# Autodesk Inventor assembly: 000-base_wheel-v2
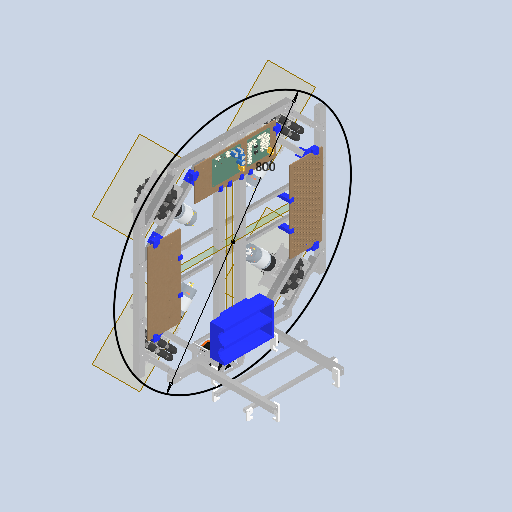
[picture p0: Inventor's stored thumbnail of the model, 512x512]
Saved by Autodesk Inventor 2025.2 (Build 292293000, 293)
## iProperties
Created: 2025-01-06
Part Number: 000-base_wheel-v2
Document SubType Name: Assembly
Designer: haruy
Mass: 4431.15 g
Surface Area: 15153.5 cm^2
Volume: 1600.59 cm^3
Density: 2.76846 g/cm^3
Author: haruy
## Documents named in this file (61)
- C:\Users\haruy\Documents\ロボコン\NHK2025\cad\nagahisa\base_weel\000-base_wheel-v2.iam
- C:\Users\haruy\Documents\ロボコン\NHK2025\cad\nagahisa\base_weel\base_weel-v2-ASP-Base.ipt
- C:\Users\haruy\Documents\ロボコン\NHK2025\cad\nagahisa\base_weel\takagi_weel\Workspaces\作業スペース\takagi\omuni_wheel_ver3.0\parts\omu_al_jo_1.ipt
- C:\Users\haruy\Documents\ロボコン\NHK2025\cad\nagahisa\base_weel\takagi_weel\Workspaces\作業スペース\takagi\omuni_wheel_ver3.0\parts\omu_al_jo_3.ipt
- C:\Users\haruy\Documents\ロボコン\NHK2025\cad\nagahisa\base_weel\takagi_weel\Workspaces\作業スペース\takagi\omuni_wheel_ver3.0\parts\frequently used parts\モーター\RS775\rs775_4.iam
- C:\Users\haruy\Documents\ロボコン\NHK2025\cad\nagahisa\base_weel\takagi_weel\Workspaces\作業スペース\takagi\omuni_wheel_ver3.0\parts\frequently used parts\セットカラー\SSCSP12-10\SSCSP12-10.iam
- C:\Users\haruy\Documents\ロボコン\NHK2025\cad\nagahisa\base_weel\takagi_weel\Workspaces\作業スペース\takagi\omuni_wheel_ver3.0\parts\omu_al_jo_2.ipt
- C:\Users\haruy\Documents\ロボコン\NHK2025\cad\nagahisa\base_weel\takagi_weel\Workspaces\作業スペース\takagi\omuni_wheel_ver3.0\parts\omu_sh_jo_2.ipt
- C:\Users\haruy\Documents\ロボコン\NHK2025\cad\nagahisa\base_weel\takagi_weel\Workspaces\作業スペース\takagi\omuni_wheel_ver3.0\parts\omu_sh_jo_3.ipt
- C:\Users\haruy\Documents\ロボコン\NHK2025\cad\nagahisa\base_weel\takagi_weel\Workspaces\作業スペース\takagi\omuni_wheel_ver3.0\parts\frequently used parts\ベアリング\B6201ZZNR\bearingB6201ZZNR.ipt
- C:\Users\haruy\Documents\ロボコン\NHK2025\cad\nagahisa\base_weel\takagi_weel\Workspaces\作業スペース\takagi\omuni_wheel_ver3.0\parts\frequently used parts\タイヤ\omni wheel\100mm wheel\100mm omuniwheel_MIR1.iam
- C:\Users\haruy\Documents\ロボコン\NHK2025\cad\nagahisa\base_weel\takagi_weel\Workspaces\作業スペース\takagi\omuni_wheel_ver3.0\parts\omu_al_jo_1_MIR2.ipt
- C:\Users\haruy\Documents\ロボコン\NHK2025\cad\nagahisa\base_weel\takagi_weel\Workspaces\作業スペース\takagi\omuni_wheel_ver3.0\parts\omu_al_jo_3_MIR2.ipt
- C:\Users\haruy\Documents\ロボコン\NHK2025\cad\nagahisa\base_weel\takagi_weel\Workspaces\作業スペース\takagi\omuni_wheel_ver3.0\parts\frequently used parts\モーター\RS775\rs775_4_MIR2.iam
- C:\Users\haruy\Documents\ロボコン\NHK2025\cad\nagahisa\base_weel\takagi_weel\Workspaces\作業スペース\takagi\omuni_wheel_ver3.0\parts\frequently used parts\セットカラー\SSCSP12-10\SSCSP12-10_MIR2.iam
- C:\Users\haruy\Documents\ロボコン\NHK2025\cad\nagahisa\base_weel\takagi_weel\Workspaces\作業スペース\takagi\omuni_wheel_ver3.0\parts\omu_al_jo_2_MIR2.ipt
- C:\Users\haruy\Documents\ロボコン\NHK2025\cad\nagahisa\base_weel\takagi_weel\Workspaces\作業スペース\takagi\omuni_wheel_ver3.0\parts\omu_sh_jo_2_MIR2.ipt
- C:\Users\haruy\Documents\ロボコン\NHK2025\cad\nagahisa\base_weel\takagi_weel\Workspaces\作業スペース\takagi\omuni_wheel_ver3.0\parts\omu_sh_jo_3_MIR2.ipt
- C:\Users\haruy\Documents\ロボコン\NHK2025\cad\nagahisa\base_weel\takagi_weel\Workspaces\作業スペース\takagi\omuni_wheel_ver3.0\parts\frequently used parts\ベアリング\B6201ZZNR\bearingB6201ZZNR_MIR2.ipt
- C:\Users\haruy\Documents\ロボコン\NHK2025\cad\nagahisa\base_weel\takagi_weel\Workspaces\作業スペース\takagi\omuni_wheel_ver3.0\parts\frequently used parts\タイヤ\omni wheel\100mm wheel\100mm omuniwheel_MIR1_MIR.iam
- C:\Users\haruy\Documents\ロボコン\NHK2025\cad\nagahisa\base_weel\takagi_weel\Workspaces\作業スペース\takagi\omuni_wheel_ver3.0\parts\omu_al_jo_1_MIR3.ipt
- C:\Users\haruy\Documents\ロボコン\NHK2025\cad\nagahisa\base_weel\takagi_weel\Workspaces\作業スペース\takagi\omuni_wheel_ver3.0\parts\omu_al_jo_3_MIR3.ipt
- C:\Users\haruy\Documents\ロボコン\NHK2025\cad\nagahisa\base_weel\takagi_weel\Workspaces\作業スペース\takagi\omuni_wheel_ver3.0\parts\frequently used parts\モーター\RS775\rs775_4_MIR3.iam
- C:\Users\haruy\Documents\ロボコン\NHK2025\cad\nagahisa\base_weel\takagi_weel\Workspaces\作業スペース\takagi\omuni_wheel_ver3.0\parts\frequently used parts\セットカラー\SSCSP12-10\SSCSP12-10_MIR3.iam
- C:\Users\haruy\Documents\ロボコン\NHK2025\cad\nagahisa\base_weel\takagi_weel\Workspaces\作業スペース\takagi\omuni_wheel_ver3.0\parts\omu_al_jo_2_MIR3.ipt
- C:\Users\haruy\Documents\ロボコン\NHK2025\cad\nagahisa\base_weel\takagi_weel\Workspaces\作業スペース\takagi\omuni_wheel_ver3.0\parts\omu_sh_jo_2_MIR3.ipt
- C:\Users\haruy\Documents\ロボコン\NHK2025\cad\nagahisa\base_weel\takagi_weel\Workspaces\作業スペース\takagi\omuni_wheel_ver3.0\parts\omu_sh_jo_3_MIR3.ipt
- C:\Users\haruy\Documents\ロボコン\NHK2025\cad\nagahisa\base_weel\takagi_weel\Workspaces\作業スペース\takagi\omuni_wheel_ver3.0\parts\frequently used parts\ベアリング\B6201ZZNR\bearingB6201ZZNR_MIR3.ipt
- C:\Users\haruy\Documents\ロボコン\NHK2025\cad\nagahisa\base_weel\takagi_weel\Workspaces\作業スペース\takagi\omuni_wheel_ver3.0\parts\frequently used parts\タイヤ\omni wheel\100mm wheel\100mm omuniwheel_MIR1_MIR1.iam
- C:\Users\haruy\Documents\ロボコン\NHK2025\cad\nagahisa\base_weel\takagi_weel\Workspaces\作業スペース\takagi\omuni_wheel_ver3.0\parts\omu_al_jo_1_MIR2_MIR.ipt
- C:\Users\haruy\Documents\ロボコン\NHK2025\cad\nagahisa\base_weel\takagi_weel\Workspaces\作業スペース\takagi\omuni_wheel_ver3.0\parts\omu_al_jo_3_MIR2_MIR.ipt
- C:\Users\haruy\Documents\ロボコン\NHK2025\cad\nagahisa\base_weel\takagi_weel\Workspaces\作業スペース\takagi\omuni_wheel_ver3.0\parts\frequently used parts\モーター\RS775\rs775_4_MIR2_MIR.iam
- C:\Users\haruy\Documents\ロボコン\NHK2025\cad\nagahisa\base_weel\takagi_weel\Workspaces\作業スペース\takagi\omuni_wheel_ver3.0\parts\frequently used parts\セットカラー\SSCSP12-10\SSCSP12-10_MIR2_MIR.iam
- C:\Users\haruy\Documents\ロボコン\NHK2025\cad\nagahisa\base_weel\takagi_weel\Workspaces\作業スペース\takagi\omuni_wheel_ver3.0\parts\omu_al_jo_2_MIR2_MIR.ipt
- C:\Users\haruy\Documents\ロボコン\NHK2025\cad\nagahisa\base_weel\takagi_weel\Workspaces\作業スペース\takagi\omuni_wheel_ver3.0\parts\omu_sh_jo_2_MIR2_MIR.ipt
- C:\Users\haruy\Documents\ロボコン\NHK2025\cad\nagahisa\base_weel\takagi_weel\Workspaces\作業スペース\takagi\omuni_wheel_ver3.0\parts\omu_sh_jo_3_MIR2_MIR.ipt
- C:\Users\haruy\Documents\ロボコン\NHK2025\cad\nagahisa\base_weel\takagi_weel\Workspaces\作業スペース\takagi\omuni_wheel_ver3.0\parts\frequently used parts\ベアリング\B6201ZZNR\bearingB6201ZZNR_MIR2_MIR.ipt
- C:\Users\haruy\Documents\ロボコン\NHK2025\cad\nagahisa\base_weel\takagi_weel\Workspaces\作業スペース\takagi\omuni_wheel_ver3.0\parts\frequently used parts\タイヤ\omni wheel\100mm wheel\100mm omuniwheel_MIR1_MIR_MIR.iam
- C:\Users\haruy\Documents\ロボコン\NHK2025\cad\nagahisa\base_weel\base_weel-v2-Plate-3.ipt
- C:\Users\haruy\Documents\ロボコン\NHK2025\cad\nagahisa\base_weel\base_weel-v2-Plate-3_MIR.ipt
- C:\Users\haruy\Documents\ロボコン\NHK2025\cad\nagahisa\base_weel\base_weel-v2-Plate-3_MIR1.ipt
- C:\Users\haruy\Documents\ロボコン\NHK2025\cad\nagahisa\base_weel\base_weel-v2-Plate-3_MIR_MIR.ipt
- C:\Users\haruy\Documents\ロボコン\NHK2025\cad\nagahisa\base_weel\base_weel-v2-Plate-4.ipt
- C:\Users\haruy\Documents\ロボコン\NHK2025\cad\nagahisa\base_weel\base_weel-v2-Plate-5.ipt
- C:\Users\haruy\Documents\ロボコン\NHK2025\cad\000_parts\センサー\LiDAR_true.iam
- C:\Users\haruy\Documents\ロボコン\NHK2025\cad\nagahisa\base_weel\base_weel-v1-Shaft-lider-spesa.ipt
- C:\Users\haruy\Documents\ロボコン\NHK2025\cad\nagahisa\base_weel\base_weel-v2-Plate-6.ipt
- C:\Users\haruy\Documents\ロボコン\NHK2025\cad\nagahisa\base_weel\base_weel-v2-Plate-7.ipt
- C:\Users\haruy\Documents\ロボコン\NHK2025\cad\nagahisa\base_weel\base_weel-v2-3DP-C-F-1.ipt
- C:\Users\haruy\Documents\ロボコン\NHK2025\cad\nagahisa\base_weel\base_weel-v2-3DP-C-F-1_MIR.ipt
- C:\Users\haruy\Documents\ロボコン\NHK2025\cad\nagahisa\base_weel\base_weel-v2-MDF-1.ipt
- C:\Users\haruy\Documents\ロボコン\NHK2025\cad\000_parts\回路関連\DCMD_Controller.ipt
- C:\Users\haruy\Documents\ロボコン\NHK2025\cad\000_parts\回路関連\mbed_Board.ipt
- C:\Users\haruy\Documents\ロボコン\NHK2025\cad\nagahisa\base_weel\base_weel-v2-MDF-2.ipt
- C:\Users\haruy\Documents\ロボコン\NHK2025\cad\nagahisa\base_weel\roja-v1-3DP-lipo-box.ipt
- C:\Users\haruy\Documents\ロボコン\NHK2025\cad\nagahisa\base_weel\base_weel-v2-Plate-8.ipt
- C:\Users\haruy\Documents\ロボコン\NHK2025\cad\nagahisa\base_weel\base_weel-v2-POM-pc-F-1.ipt
- C:\Users\haruy\Documents\ロボコン\NHK2025\cad\nagahisa\base_weel\base_weel-v2-POM-pc-F-2.ipt
- C:\Users\haruy\Documents\ロボコン\NHK2025\cad\nagahisa\base_weel\base_weel-v2-MDF-3.ipt
- C:\Users\haruy\Documents\ロボコン\NHK2025\cad\nagahisa\base_weel\base_weel-v2-3DP-C-F-2.ipt
- C:\Users\haruy\Documents\ロボコン\NHK2025\cad\nagahisa\base_weel\base_weel-v2-3DP-C-F-3.ipt
## Components (112 placed, 60 different names)
1. base_weel-v2-ASP-Base:1 — 挿入:12, 挿入:13, 角度:1, フラッシュ:1, 挿入:35, 挿入:36, 挿入:48, 挿入:49, 挿入:50, 挿入:51, 挿入:74, 挿入:75, 挿入:76, 挿入:77, 挿入:78, 挿入:79, 挿入:80, 挿入:81, 挿入:82, 挿入:83, 挿入:84, 挿入:85, 挿入:86, 挿入:87, 挿入:88, 挿入:89, 挿入:90, 挿入:91, 挿入:92, 挿入:93, 挿入:94, 挿入:95, 挿入:96, 挿入:97, 挿入:98, 挿入:99, 挿入:100, 挿入:101, 挿入:102, 挿入:103, 挿入:104, 挿入:105, 挿入:106, 挿入:107, 挿入:108, 挿入:109, 挿入:110, 挿入:111, 挿入:112, 挿入:113, 挿入:114, 挿入:115, 挿入:116, 挿入:117, 挿入:118, 挿入:119, 挿入:120, 挿入:121, 挿入:122, フラッシュ:2, 挿入:129, 挿入:130, 角度:4, 角度:5, 角度:6, 挿入:149, 挿入:151, 挿入:152, 挿入:153, 挿入:154, 挿入:155, 挿入:156, 挿入:157, 挿入:158, 挿入:159, 挿入:160, 挿入:161, 挿入:162, 挿入:163, 挿入:164, 挿入:165, 挿入:166, 挿入:167, 挿入:168, 挿入:169, 挿入:170, 挿入:171, 挿入:172, 挿入:173, 挿入:174, 挿入:185, 挿入:186, 挿入:187, 挿入:188, 挿入:189, 挿入:190, 挿入:191, 挿入:192, 挿入:193, 挿入:194, 挿入:195, 挿入:196, 挿入:197, 挿入:198, 挿入:199, 挿入:200, 挿入:201, 挿入:202, メイト:19, 挿入:203, 挿入:204, メイト:20, 挿入:205, 挿入:206, メイト:21, 挿入:216
2. omu_al_jo_1:1 — 挿入:20, 挿入:21, 挿入:23, 挿入:35, 挿入:36
3. omu_al_jo_3:1 — 挿入:12, 挿入:13, 挿入:22
4. rs775_4:1 [sub-assembly]
5. SSCSP12-10:1 [sub-assembly]
6. omu_al_jo_2:1
7. omu_sh_jo_2:1
8. omu_sh_jo_3:1 — 挿入:21
9. omu_sh_jo_3:2
10. omu_sh_jo_3:3 — 挿入:20
11. omu_sh_jo_3:4
12. bearingB6201ZZNR:1 — 挿入:23, 挿入:24
13. bearingB6201ZZNR:2 — 挿入:22
14. 100mm omuniwheel_MIR1:1 [sub-assembly] — 角度:1, 挿入:24
15. omu_al_jo_1_MIR2:1 — 挿入:39, 挿入:42, 挿入:45, 挿入:50, 挿入:51
16. omu_al_jo_3_MIR2:1 — 挿入:46, 挿入:48, 挿入:49
17. rs775_4_MIR2:1 [sub-assembly] — メイト:7, 挿入:37, 挿入:38, メイト:8, メイト:9
18. SSCSP12-10_MIR2:1 [sub-assembly] — メイト:7, メイト:10
19. omu_al_jo_2_MIR2:1 — 挿入:37, 挿入:38, 挿入:40, 挿入:41, 挿入:43, 挿入:44
20. omu_sh_jo_2_MIR2:1 — メイト:8, メイト:9, メイト:10
21. omu_sh_jo_3_MIR2:1 — 挿入:39, 挿入:40
22. omu_sh_jo_3_MIR2:2 — 挿入:41
23. omu_sh_jo_3_MIR2:3 — 挿入:42, 挿入:43
24. omu_sh_jo_3_MIR2:4 — 挿入:44
25. bearingB6201ZZNR_MIR2:1 — 挿入:45, 挿入:47
26. bearingB6201ZZNR_MIR2:2 — 挿入:46
27. 100mm omuniwheel_MIR1_MIR:1 [sub-assembly] — 挿入:47, 角度:4
28. omu_al_jo_1_MIR3:1 — 挿入:54, 挿入:57, 挿入:60, 挿入:74, 挿入:75
29. omu_al_jo_3_MIR3:1 — 挿入:61, 挿入:76, 挿入:77
30. rs775_4_MIR3:1 [sub-assembly] — メイト:11, 挿入:52, 挿入:53, メイト:12, メイト:13
31. SSCSP12-10_MIR3:1 [sub-assembly] — メイト:11, メイト:14
32. omu_al_jo_2_MIR3:1 — 挿入:52, 挿入:53, 挿入:55, 挿入:56, 挿入:58, 挿入:59
33. omu_sh_jo_2_MIR3:1 — メイト:12, メイト:13, メイト:14
34. omu_sh_jo_3_MIR3:1 — 挿入:54, 挿入:55
35. omu_sh_jo_3_MIR3:2 — 挿入:56
36. omu_sh_jo_3_MIR3:3 — 挿入:57, 挿入:58
37. omu_sh_jo_3_MIR3:4 — 挿入:59
38. bearingB6201ZZNR_MIR3:1 — 挿入:60, 挿入:62
39. bearingB6201ZZNR_MIR3:2 — 挿入:61
40. 100mm omuniwheel_MIR1_MIR1:1 [sub-assembly] — 挿入:62, 角度:6
41. omu_al_jo_1_MIR2_MIR:1 — 挿入:66, 挿入:69, 挿入:71, 挿入:80, 挿入:81
42. omu_al_jo_3_MIR2_MIR:1 — 挿入:72, 挿入:78, 挿入:79
43. rs775_4_MIR2_MIR:1 [sub-assembly] — メイト:15, 挿入:63, 挿入:64, メイト:17, メイト:18
44. SSCSP12-10_MIR2_MIR:1 [sub-assembly] — メイト:15, メイト:16
45. omu_al_jo_2_MIR2_MIR:1 — 挿入:63, 挿入:64, 挿入:65, 挿入:67, 挿入:68, 挿入:70
46. omu_sh_jo_2_MIR2_MIR:1 — メイト:16, メイト:17, メイト:18
47. omu_sh_jo_3_MIR2_MIR:1 — 挿入:65, 挿入:66
48. omu_sh_jo_3_MIR2_MIR:2 — 挿入:67
49. omu_sh_jo_3_MIR2_MIR:3 — 挿入:68, 挿入:69
50. omu_sh_jo_3_MIR2_MIR:4 — 挿入:70
51. bearingB6201ZZNR_MIR2_MIR:1 — 挿入:71, 挿入:73
52. bearingB6201ZZNR_MIR2_MIR:2 — 挿入:72
53. 100mm omuniwheel_MIR1_MIR_MIR:1 [sub-assembly] — 挿入:73, 角度:5
54. base_weel-v2-Plate-3:1 — 挿入:82, 挿入:84
55. base_weel-v2-Plate-3:2 — 挿入:83, 挿入:85, 挿入:86
56. base_weel-v2-Plate-3:3 — 挿入:87, 挿入:88
57. base_weel-v2-Plate-3:4 — 挿入:89, 挿入:90
58. base_weel-v2-Plate-3_MIR:1 — 挿入:95, 挿入:96
59. base_weel-v2-Plate-3_MIR:2 — 挿入:97, 挿入:98
60. base_weel-v2-Plate-3_MIR:3 — 挿入:91, 挿入:92
61. base_weel-v2-Plate-3_MIR:4 — 挿入:93, 挿入:94
62. base_weel-v2-Plate-3_MIR1:1 — 挿入:101, 挿入:102
63. base_weel-v2-Plate-3_MIR1:2 — 挿入:99, 挿入:100
64. base_weel-v2-Plate-3_MIR1:3 — 挿入:103, 挿入:104
65. base_weel-v2-Plate-3_MIR1:4 — 挿入:105, 挿入:106
66. base_weel-v2-Plate-3_MIR_MIR:1 — 挿入:113, 挿入:114
67. base_weel-v2-Plate-3_MIR_MIR:2 — 挿入:111, 挿入:112
68. base_weel-v2-Plate-3_MIR_MIR:3 — 挿入:109, 挿入:110
69. base_weel-v2-Plate-3_MIR_MIR:4 — 挿入:107, 挿入:108
70. base_weel-v2-Plate-4:1 — 挿入:116, 挿入:117
71. base_weel-v2-Plate-4:2 — 挿入:115, 挿入:118
72. base_weel-v2-Plate-4:3 — 挿入:121, 挿入:122
73. base_weel-v2-Plate-4:4 — 挿入:119, 挿入:120
74. base_weel-v2-Plate-5:1 — 挿入:123, 挿入:124, フラッシュ:2, 挿入:125, 挿入:126, 角度:2, 角度:3, 挿入:131, 挿入:132
75. LiDAR_true:1 [sub-assembly] — 挿入:123, 挿入:124
76. base_weel-v1-Shaft-lider-spesa:1 — 挿入:126, 挿入:128
77. base_weel-v1-Shaft-lider-spesa:2 — 挿入:125, 挿入:127
78. base_weel-v2-Plate-6:1 — 挿入:127, 挿入:128
79. base_weel-v2-Plate-7:1 — 挿入:129, 角度:2, 挿入:131, 挿入:132
80. base_weel-v2-Plate-7:2 — 挿入:130, 角度:3
81. base_weel-v2-3DP-C-F-1:1 — 挿入:138, 挿入:201, 挿入:202
82. base_weel-v2-3DP-C-F-1_MIR:1 — 挿入:137, メイト:19
83. base_weel-v2-MDF-1:1 — 挿入:137, 挿入:138, 挿入:139, 挿入:140, 挿入:141, 挿入:142
84. DCMD_Controller:1 — 挿入:141, 挿入:142
85. mbed_Board:1 — 挿入:139, 挿入:140
86. base_weel-v2-3DP-C-F-1:2 — 挿入:148, 挿入:203, 挿入:204
87. base_weel-v2-3DP-C-F-1_MIR:2 — 挿入:147, メイト:20
88. base_weel-v2-MDF-2:1 — 挿入:147, 挿入:148
89. roja-v1-3DP-lipo-box:1 — 挿入:149, 挿入:216
90. base_weel-v2-Plate-8:1 — 挿入:151, 挿入:152
91. base_weel-v2-Plate-8:2 — 挿入:153, 挿入:154
92. base_weel-v2-Plate-8:3 — 挿入:155, 挿入:156
93. base_weel-v2-Plate-8:4 — 挿入:157, 挿入:158
94. base_weel-v2-POM-pc-F-1:1 — 挿入:159, 挿入:160
95. base_weel-v2-POM-pc-F-1:2 — 挿入:165, 挿入:166
96. base_weel-v2-POM-pc-F-1:3 — 挿入:161, 挿入:162
97. base_weel-v2-POM-pc-F-1:4 — 挿入:163, 挿入:164
98. base_weel-v2-POM-pc-F-2:1 — 挿入:169, 挿入:170
99. base_weel-v2-POM-pc-F-2:2 — 挿入:167, 挿入:168
100. base_weel-v2-POM-pc-F-2:3 — 挿入:173, 挿入:174
101. base_weel-v2-POM-pc-F-2:4 — 挿入:171, 挿入:172
102. base_weel-v2-3DP-C-F-1:3 — 挿入:179, 挿入:205, 挿入:206
103. base_weel-v2-3DP-C-F-1_MIR:3 — 挿入:180, メイト:21
104. base_weel-v2-MDF-3:1 — 挿入:179, 挿入:180
105. base_weel-v2-3DP-C-F-2:1 — 挿入:185, 挿入:186
106. base_weel-v2-3DP-C-F-2:2 — 挿入:187, 挿入:188
107. base_weel-v2-3DP-C-F-2:3 — 挿入:189, 挿入:190
108. base_weel-v2-3DP-C-F-2:4 — 挿入:191, 挿入:192
109. base_weel-v2-3DP-C-F-3:1 — 挿入:193, 挿入:194
110. base_weel-v2-3DP-C-F-3:2 — 挿入:195, 挿入:196
111. base_weel-v2-3DP-C-F-3:3 — 挿入:199, 挿入:200
112. base_weel-v2-3DP-C-F-3:4 — 挿入:197, 挿入:198
## Relationships (196: Insert 169, Mate 19, Angle 6, Flush 2)
- 挿入:12 [Insert]: base_weel-v2-ASP-Base:1 ↔ omu_al_jo_3:1
- 挿入:13 [Insert]: base_weel-v2-ASP-Base:1 ↔ omu_al_jo_3:1
- [Mate] (5 mm): rs775_4:1 ↔ SSCSP12-10:1
- [Insert]: rs775_4:1 ↔ omu_al_jo_2:1
- [Insert]: rs775_4:1 ↔ omu_al_jo_2:1
- [Mate]: SSCSP12-10:1 ↔ omu_sh_jo_2:1
- [Mate]: rs775_4:1 ↔ omu_sh_jo_2:1
- [Mate]: rs775_4:1 ↔ omu_sh_jo_2:1
- [Insert]: omu_al_jo_2:1 ↔ omu_sh_jo_3:1
- [Insert]: omu_al_jo_2:1 ↔ omu_sh_jo_3:4
- [Insert]: omu_al_jo_2:1 ↔ omu_sh_jo_3:2
- [Insert]: omu_al_jo_2:1 ↔ omu_sh_jo_3:3
- 挿入:20 [Insert]: omu_al_jo_1:1 ↔ omu_sh_jo_3:3
- 挿入:21 [Insert]: omu_al_jo_1:1 ↔ omu_sh_jo_3:1
- 挿入:22 [Insert]: omu_al_jo_3:1 ↔ bearingB6201ZZNR:2
- 挿入:23 [Insert]: omu_al_jo_1:1 ↔ bearingB6201ZZNR:1
- 角度:1 [Angle] (0 deg): base_weel-v2-ASP-Base:1 ↔ 100mm omuniwheel_MIR1:1
- 挿入:24 [Insert] (12 mm): bearingB6201ZZNR:1 ↔ 100mm omuniwheel_MIR1:1
- フラッシュ:1 [Flush] (17 mm): base_weel-v2-ASP-Base:1
- 挿入:35 [Insert]: base_weel-v2-ASP-Base:1 ↔ omu_al_jo_1:1
- 挿入:36 [Insert]: base_weel-v2-ASP-Base:1 ↔ omu_al_jo_1:1
- メイト:7 [Mate] (5 mm): rs775_4_MIR2:1 ↔ SSCSP12-10_MIR2:1
- 挿入:37 [Insert]: rs775_4_MIR2:1 ↔ omu_al_jo_2_MIR2:1
- 挿入:38 [Insert]: rs775_4_MIR2:1 ↔ omu_al_jo_2_MIR2:1
- メイト:8 [Mate]: rs775_4_MIR2:1 ↔ omu_sh_jo_2_MIR2:1
- メイト:9 [Mate]: rs775_4_MIR2:1 ↔ omu_sh_jo_2_MIR2:1
- メイト:10 [Mate]: SSCSP12-10_MIR2:1 ↔ omu_sh_jo_2_MIR2:1
- 挿入:39 [Insert]: omu_al_jo_1_MIR2:1 ↔ omu_sh_jo_3_MIR2:1
- 挿入:40 [Insert]: omu_al_jo_2_MIR2:1 ↔ omu_sh_jo_3_MIR2:1
- 挿入:41 [Insert]: omu_al_jo_2_MIR2:1 ↔ omu_sh_jo_3_MIR2:2
- 挿入:42 [Insert]: omu_al_jo_1_MIR2:1 ↔ omu_sh_jo_3_MIR2:3
- 挿入:43 [Insert]: omu_al_jo_2_MIR2:1 ↔ omu_sh_jo_3_MIR2:3
- 挿入:44 [Insert]: omu_al_jo_2_MIR2:1 ↔ omu_sh_jo_3_MIR2:4
- 挿入:45 [Insert]: omu_al_jo_1_MIR2:1 ↔ bearingB6201ZZNR_MIR2:1
- 挿入:46 [Insert]: omu_al_jo_3_MIR2:1 ↔ bearingB6201ZZNR_MIR2:2
- 挿入:47 [Insert] (12 mm): bearingB6201ZZNR_MIR2:1 ↔ 100mm omuniwheel_MIR1_MIR:1
- 挿入:48 [Insert]: base_weel-v2-ASP-Base:1 ↔ omu_al_jo_3_MIR2:1
- 挿入:49 [Insert]: base_weel-v2-ASP-Base:1 ↔ omu_al_jo_3_MIR2:1
- 挿入:50 [Insert]: base_weel-v2-ASP-Base:1 ↔ omu_al_jo_1_MIR2:1
- 挿入:51 [Insert]: base_weel-v2-ASP-Base:1 ↔ omu_al_jo_1_MIR2:1
- メイト:11 [Mate] (5 mm): rs775_4_MIR3:1 ↔ SSCSP12-10_MIR3:1
- 挿入:52 [Insert]: rs775_4_MIR3:1 ↔ omu_al_jo_2_MIR3:1
- 挿入:53 [Insert]: rs775_4_MIR3:1 ↔ omu_al_jo_2_MIR3:1
- メイト:12 [Mate]: rs775_4_MIR3:1 ↔ omu_sh_jo_2_MIR3:1
- メイト:13 [Mate]: rs775_4_MIR3:1 ↔ omu_sh_jo_2_MIR3:1
- メイト:14 [Mate]: SSCSP12-10_MIR3:1 ↔ omu_sh_jo_2_MIR3:1
- 挿入:54 [Insert]: omu_al_jo_1_MIR3:1 ↔ omu_sh_jo_3_MIR3:1
- 挿入:55 [Insert]: omu_al_jo_2_MIR3:1 ↔ omu_sh_jo_3_MIR3:1
- 挿入:56 [Insert]: omu_al_jo_2_MIR3:1 ↔ omu_sh_jo_3_MIR3:2
- 挿入:57 [Insert]: omu_al_jo_1_MIR3:1 ↔ omu_sh_jo_3_MIR3:3
- 挿入:58 [Insert]: omu_al_jo_2_MIR3:1 ↔ omu_sh_jo_3_MIR3:3
- 挿入:59 [Insert]: omu_al_jo_2_MIR3:1 ↔ omu_sh_jo_3_MIR3:4
- 挿入:60 [Insert]: omu_al_jo_1_MIR3:1 ↔ bearingB6201ZZNR_MIR3:1
- 挿入:61 [Insert]: omu_al_jo_3_MIR3:1 ↔ bearingB6201ZZNR_MIR3:2
- 挿入:62 [Insert] (12 mm): bearingB6201ZZNR_MIR3:1 ↔ 100mm omuniwheel_MIR1_MIR1:1
- メイト:15 [Mate] (5 mm): rs775_4_MIR2_MIR:1 ↔ SSCSP12-10_MIR2_MIR:1
- 挿入:63 [Insert]: rs775_4_MIR2_MIR:1 ↔ omu_al_jo_2_MIR2_MIR:1
- 挿入:64 [Insert]: rs775_4_MIR2_MIR:1 ↔ omu_al_jo_2_MIR2_MIR:1
- メイト:16 [Mate]: SSCSP12-10_MIR2_MIR:1 ↔ omu_sh_jo_2_MIR2_MIR:1
- メイト:17 [Mate]: rs775_4_MIR2_MIR:1 ↔ omu_sh_jo_2_MIR2_MIR:1
- メイト:18 [Mate]: rs775_4_MIR2_MIR:1 ↔ omu_sh_jo_2_MIR2_MIR:1
- 挿入:65 [Insert]: omu_al_jo_2_MIR2_MIR:1 ↔ omu_sh_jo_3_MIR2_MIR:1
- 挿入:66 [Insert]: omu_al_jo_1_MIR2_MIR:1 ↔ omu_sh_jo_3_MIR2_MIR:1
- 挿入:67 [Insert]: omu_al_jo_2_MIR2_MIR:1 ↔ omu_sh_jo_3_MIR2_MIR:2
- 挿入:68 [Insert]: omu_al_jo_2_MIR2_MIR:1 ↔ omu_sh_jo_3_MIR2_MIR:3
- 挿入:69 [Insert]: omu_al_jo_1_MIR2_MIR:1 ↔ omu_sh_jo_3_MIR2_MIR:3
- 挿入:70 [Insert]: omu_al_jo_2_MIR2_MIR:1 ↔ omu_sh_jo_3_MIR2_MIR:4
- 挿入:71 [Insert]: omu_al_jo_1_MIR2_MIR:1 ↔ bearingB6201ZZNR_MIR2_MIR:1
- 挿入:72 [Insert]: omu_al_jo_3_MIR2_MIR:1 ↔ bearingB6201ZZNR_MIR2_MIR:2
- 挿入:73 [Insert] (12 mm): bearingB6201ZZNR_MIR2_MIR:1 ↔ 100mm omuniwheel_MIR1_MIR_MIR:1
- 挿入:74 [Insert]: base_weel-v2-ASP-Base:1 ↔ omu_al_jo_1_MIR3:1
- 挿入:75 [Insert]: base_weel-v2-ASP-Base:1 ↔ omu_al_jo_1_MIR3:1
- 挿入:76 [Insert]: base_weel-v2-ASP-Base:1 ↔ omu_al_jo_3_MIR3:1
- 挿入:77 [Insert]: base_weel-v2-ASP-Base:1 ↔ omu_al_jo_3_MIR3:1
- 挿入:78 [Insert]: base_weel-v2-ASP-Base:1 ↔ omu_al_jo_3_MIR2_MIR:1
- 挿入:79 [Insert]: base_weel-v2-ASP-Base:1 ↔ omu_al_jo_3_MIR2_MIR:1
- 挿入:80 [Insert]: base_weel-v2-ASP-Base:1 ↔ omu_al_jo_1_MIR2_MIR:1
- 挿入:81 [Insert]: base_weel-v2-ASP-Base:1 ↔ omu_al_jo_1_MIR2_MIR:1
- 挿入:82 [Insert]: base_weel-v2-ASP-Base:1 ↔ base_weel-v2-Plate-3:1
- 挿入:83 [Insert]: base_weel-v2-ASP-Base:1 ↔ base_weel-v2-Plate-3:2
- 挿入:84 [Insert]: base_weel-v2-ASP-Base:1 ↔ base_weel-v2-Plate-3:1
- 挿入:85 [Insert]: base_weel-v2-ASP-Base:1 ↔ base_weel-v2-Plate-3:2
- 挿入:86 [Insert]: base_weel-v2-ASP-Base:1 ↔ base_weel-v2-Plate-3:2
- 挿入:87 [Insert]: base_weel-v2-ASP-Base:1 ↔ base_weel-v2-Plate-3:3
- 挿入:88 [Insert]: base_weel-v2-ASP-Base:1 ↔ base_weel-v2-Plate-3:3
- 挿入:89 [Insert]: base_weel-v2-ASP-Base:1 ↔ base_weel-v2-Plate-3:4
- 挿入:90 [Insert]: base_weel-v2-ASP-Base:1 ↔ base_weel-v2-Plate-3:4
- 挿入:91 [Insert]: base_weel-v2-ASP-Base:1 ↔ base_weel-v2-Plate-3_MIR:3
- 挿入:92 [Insert]: base_weel-v2-ASP-Base:1 ↔ base_weel-v2-Plate-3_MIR:3
- 挿入:93 [Insert]: base_weel-v2-ASP-Base:1 ↔ base_weel-v2-Plate-3_MIR:4
- 挿入:94 [Insert]: base_weel-v2-ASP-Base:1 ↔ base_weel-v2-Plate-3_MIR:4
- 挿入:95 [Insert]: base_weel-v2-ASP-Base:1 ↔ base_weel-v2-Plate-3_MIR:1
- 挿入:96 [Insert]: base_weel-v2-ASP-Base:1 ↔ base_weel-v2-Plate-3_MIR:1
- 挿入:97 [Insert]: base_weel-v2-ASP-Base:1 ↔ base_weel-v2-Plate-3_MIR:2
- 挿入:98 [Insert]: base_weel-v2-ASP-Base:1 ↔ base_weel-v2-Plate-3_MIR:2
- 挿入:99 [Insert]: base_weel-v2-ASP-Base:1 ↔ base_weel-v2-Plate-3_MIR1:2
- 挿入:100 [Insert]: base_weel-v2-ASP-Base:1 ↔ base_weel-v2-Plate-3_MIR1:2
- 挿入:101 [Insert]: base_weel-v2-ASP-Base:1 ↔ base_weel-v2-Plate-3_MIR1:1
- 挿入:102 [Insert]: base_weel-v2-ASP-Base:1 ↔ base_weel-v2-Plate-3_MIR1:1
- 挿入:103 [Insert]: base_weel-v2-ASP-Base:1 ↔ base_weel-v2-Plate-3_MIR1:3
- 挿入:104 [Insert]: base_weel-v2-ASP-Base:1 ↔ base_weel-v2-Plate-3_MIR1:3
- 挿入:105 [Insert]: base_weel-v2-ASP-Base:1 ↔ base_weel-v2-Plate-3_MIR1:4
- 挿入:106 [Insert]: base_weel-v2-ASP-Base:1 ↔ base_weel-v2-Plate-3_MIR1:4
- 挿入:107 [Insert]: base_weel-v2-ASP-Base:1 ↔ base_weel-v2-Plate-3_MIR_MIR:4
- 挿入:108 [Insert]: base_weel-v2-ASP-Base:1 ↔ base_weel-v2-Plate-3_MIR_MIR:4
- 挿入:109 [Insert]: base_weel-v2-ASP-Base:1 ↔ base_weel-v2-Plate-3_MIR_MIR:3
- 挿入:110 [Insert]: base_weel-v2-ASP-Base:1 ↔ base_weel-v2-Plate-3_MIR_MIR:3
- 挿入:111 [Insert]: base_weel-v2-ASP-Base:1 ↔ base_weel-v2-Plate-3_MIR_MIR:2
- 挿入:112 [Insert]: base_weel-v2-ASP-Base:1 ↔ base_weel-v2-Plate-3_MIR_MIR:2
- 挿入:113 [Insert]: base_weel-v2-ASP-Base:1 ↔ base_weel-v2-Plate-3_MIR_MIR:1
- 挿入:114 [Insert]: base_weel-v2-ASP-Base:1 ↔ base_weel-v2-Plate-3_MIR_MIR:1
- 挿入:115 [Insert]: base_weel-v2-ASP-Base:1 ↔ base_weel-v2-Plate-4:2
- 挿入:116 [Insert]: base_weel-v2-ASP-Base:1 ↔ base_weel-v2-Plate-4:1
- 挿入:117 [Insert]: base_weel-v2-ASP-Base:1 ↔ base_weel-v2-Plate-4:1
- 挿入:118 [Insert]: base_weel-v2-ASP-Base:1 ↔ base_weel-v2-Plate-4:2
- 挿入:119 [Insert]: base_weel-v2-ASP-Base:1 ↔ base_weel-v2-Plate-4:4
- 挿入:120 [Insert]: base_weel-v2-ASP-Base:1 ↔ base_weel-v2-Plate-4:4
- 挿入:121 [Insert]: base_weel-v2-ASP-Base:1 ↔ base_weel-v2-Plate-4:3
- 挿入:122 [Insert]: base_weel-v2-ASP-Base:1 ↔ base_weel-v2-Plate-4:3
- 挿入:123 [Insert]: base_weel-v2-Plate-5:1 ↔ LiDAR_true:1
- 挿入:124 [Insert]: base_weel-v2-Plate-5:1 ↔ LiDAR_true:1
- フラッシュ:2 [Flush]: base_weel-v2-ASP-Base:1 ↔ base_weel-v2-Plate-5:1
- 挿入:125 [Insert]: base_weel-v2-Plate-5:1 ↔ base_weel-v1-Shaft-lider-spesa:2
- 挿入:126 [Insert]: base_weel-v2-Plate-5:1 ↔ base_weel-v1-Shaft-lider-spesa:1
- 挿入:127 [Insert]: base_weel-v1-Shaft-lider-spesa:2 ↔ base_weel-v2-Plate-6:1
- 挿入:128 [Insert]: base_weel-v1-Shaft-lider-spesa:1 ↔ base_weel-v2-Plate-6:1
- 挿入:129 [Insert]: base_weel-v2-ASP-Base:1 ↔ base_weel-v2-Plate-7:1
- 角度:2 [Angle] (0 deg): base_weel-v2-Plate-5:1 ↔ base_weel-v2-Plate-7:1
- 挿入:130 [Insert]: base_weel-v2-ASP-Base:1 ↔ base_weel-v2-Plate-7:2
- 角度:3 [Angle] (180 deg): base_weel-v2-Plate-5:1 ↔ base_weel-v2-Plate-7:2
- 挿入:131 [Insert]: base_weel-v2-Plate-5:1 ↔ base_weel-v2-Plate-7:1
- 挿入:132 [Insert]: base_weel-v2-Plate-5:1 ↔ base_weel-v2-Plate-7:1
- 角度:4 [Angle] (180 deg): base_weel-v2-ASP-Base:1 ↔ 100mm omuniwheel_MIR1_MIR:1
- 角度:5 [Angle] (180 deg): base_weel-v2-ASP-Base:1 ↔ 100mm omuniwheel_MIR1_MIR_MIR:1
- 角度:6 [Angle] (180 deg): base_weel-v2-ASP-Base:1 ↔ 100mm omuniwheel_MIR1_MIR1:1
- 挿入:137 [Insert]: base_weel-v2-3DP-C-F-1_MIR:1 ↔ base_weel-v2-MDF-1:1
- 挿入:138 [Insert]: base_weel-v2-3DP-C-F-1:1 ↔ base_weel-v2-MDF-1:1
- 挿入:139 [Insert]: base_weel-v2-MDF-1:1 ↔ mbed_Board:1
- 挿入:140 [Insert]: base_weel-v2-MDF-1:1 ↔ mbed_Board:1
- 挿入:141 [Insert]: base_weel-v2-MDF-1:1 ↔ DCMD_Controller:1
- 挿入:142 [Insert]: base_weel-v2-MDF-1:1 ↔ DCMD_Controller:1
- 挿入:147 [Insert]: base_weel-v2-3DP-C-F-1_MIR:2 ↔ base_weel-v2-MDF-2:1
- 挿入:148 [Insert]: base_weel-v2-3DP-C-F-1:2 ↔ base_weel-v2-MDF-2:1
- 挿入:149 [Insert]: base_weel-v2-ASP-Base:1 ↔ roja-v1-3DP-lipo-box:1
- 挿入:151 [Insert]: base_weel-v2-ASP-Base:1 ↔ base_weel-v2-Plate-8:1
- 挿入:152 [Insert]: base_weel-v2-ASP-Base:1 ↔ base_weel-v2-Plate-8:1
- 挿入:153 [Insert]: base_weel-v2-ASP-Base:1 ↔ base_weel-v2-Plate-8:2
- 挿入:154 [Insert]: base_weel-v2-ASP-Base:1 ↔ base_weel-v2-Plate-8:2
- 挿入:155 [Insert]: base_weel-v2-ASP-Base:1 ↔ base_weel-v2-Plate-8:3
- 挿入:156 [Insert]: base_weel-v2-ASP-Base:1 ↔ base_weel-v2-Plate-8:3
- 挿入:157 [Insert]: base_weel-v2-ASP-Base:1 ↔ base_weel-v2-Plate-8:4
- 挿入:158 [Insert]: base_weel-v2-ASP-Base:1 ↔ base_weel-v2-Plate-8:4
- 挿入:159 [Insert]: base_weel-v2-ASP-Base:1 ↔ base_weel-v2-POM-pc-F-1:1
- 挿入:160 [Insert]: base_weel-v2-ASP-Base:1 ↔ base_weel-v2-POM-pc-F-1:1
- 挿入:161 [Insert]: base_weel-v2-ASP-Base:1 ↔ base_weel-v2-POM-pc-F-1:3
- 挿入:162 [Insert]: base_weel-v2-ASP-Base:1 ↔ base_weel-v2-POM-pc-F-1:3
- 挿入:163 [Insert]: base_weel-v2-ASP-Base:1 ↔ base_weel-v2-POM-pc-F-1:4
- 挿入:164 [Insert]: base_weel-v2-ASP-Base:1 ↔ base_weel-v2-POM-pc-F-1:4
- 挿入:165 [Insert]: base_weel-v2-ASP-Base:1 ↔ base_weel-v2-POM-pc-F-1:2
- 挿入:166 [Insert]: base_weel-v2-ASP-Base:1 ↔ base_weel-v2-POM-pc-F-1:2
- 挿入:167 [Insert]: base_weel-v2-ASP-Base:1 ↔ base_weel-v2-POM-pc-F-2:2
- 挿入:168 [Insert]: base_weel-v2-ASP-Base:1 ↔ base_weel-v2-POM-pc-F-2:2
- 挿入:169 [Insert]: base_weel-v2-ASP-Base:1 ↔ base_weel-v2-POM-pc-F-2:1
- 挿入:170 [Insert]: base_weel-v2-ASP-Base:1 ↔ base_weel-v2-POM-pc-F-2:1
- 挿入:171 [Insert]: base_weel-v2-ASP-Base:1 ↔ base_weel-v2-POM-pc-F-2:4
- 挿入:172 [Insert]: base_weel-v2-ASP-Base:1 ↔ base_weel-v2-POM-pc-F-2:4
- 挿入:173 [Insert]: base_weel-v2-ASP-Base:1 ↔ base_weel-v2-POM-pc-F-2:3
- 挿入:174 [Insert]: base_weel-v2-ASP-Base:1 ↔ base_weel-v2-POM-pc-F-2:3
- 挿入:179 [Insert]: base_weel-v2-3DP-C-F-1:3 ↔ base_weel-v2-MDF-3:1
- 挿入:180 [Insert]: base_weel-v2-3DP-C-F-1_MIR:3 ↔ base_weel-v2-MDF-3:1
- 挿入:185 [Insert]: base_weel-v2-ASP-Base:1 ↔ base_weel-v2-3DP-C-F-2:1
- 挿入:186 [Insert]: base_weel-v2-ASP-Base:1 ↔ base_weel-v2-3DP-C-F-2:1
- 挿入:187 [Insert]: base_weel-v2-ASP-Base:1 ↔ base_weel-v2-3DP-C-F-2:2
- 挿入:188 [Insert]: base_weel-v2-ASP-Base:1 ↔ base_weel-v2-3DP-C-F-2:2
- 挿入:189 [Insert]: base_weel-v2-ASP-Base:1 ↔ base_weel-v2-3DP-C-F-2:3
- 挿入:190 [Insert]: base_weel-v2-ASP-Base:1 ↔ base_weel-v2-3DP-C-F-2:3
- 挿入:191 [Insert]: base_weel-v2-ASP-Base:1 ↔ base_weel-v2-3DP-C-F-2:4
- 挿入:192 [Insert]: base_weel-v2-ASP-Base:1 ↔ base_weel-v2-3DP-C-F-2:4
- 挿入:193 [Insert]: base_weel-v2-ASP-Base:1 ↔ base_weel-v2-3DP-C-F-3:1
- 挿入:194 [Insert]: base_weel-v2-ASP-Base:1 ↔ base_weel-v2-3DP-C-F-3:1
- 挿入:195 [Insert]: base_weel-v2-ASP-Base:1 ↔ base_weel-v2-3DP-C-F-3:2
- 挿入:196 [Insert]: base_weel-v2-ASP-Base:1 ↔ base_weel-v2-3DP-C-F-3:2
- 挿入:197 [Insert]: base_weel-v2-ASP-Base:1 ↔ base_weel-v2-3DP-C-F-3:4
- 挿入:198 [Insert]: base_weel-v2-ASP-Base:1 ↔ base_weel-v2-3DP-C-F-3:4
- 挿入:199 [Insert]: base_weel-v2-ASP-Base:1 ↔ base_weel-v2-3DP-C-F-3:3
- 挿入:200 [Insert]: base_weel-v2-ASP-Base:1 ↔ base_weel-v2-3DP-C-F-3:3
- 挿入:201 [Insert]: base_weel-v2-ASP-Base:1 ↔ base_weel-v2-3DP-C-F-1:1
- 挿入:202 [Insert]: base_weel-v2-ASP-Base:1 ↔ base_weel-v2-3DP-C-F-1:1
- メイト:19 [Mate] (0.2 mm): base_weel-v2-ASP-Base:1 ↔ base_weel-v2-3DP-C-F-1_MIR:1
- 挿入:203 [Insert]: base_weel-v2-ASP-Base:1 ↔ base_weel-v2-3DP-C-F-1:2
- 挿入:204 [Insert]: base_weel-v2-ASP-Base:1 ↔ base_weel-v2-3DP-C-F-1:2
- メイト:20 [Mate] (0.2 mm): base_weel-v2-ASP-Base:1 ↔ base_weel-v2-3DP-C-F-1_MIR:2
- 挿入:205 [Insert]: base_weel-v2-ASP-Base:1 ↔ base_weel-v2-3DP-C-F-1:3
- 挿入:206 [Insert]: base_weel-v2-ASP-Base:1 ↔ base_weel-v2-3DP-C-F-1:3
- メイト:21 [Mate]: base_weel-v2-ASP-Base:1 ↔ base_weel-v2-3DP-C-F-1_MIR:3
- 挿入:216 [Insert]: base_weel-v2-ASP-Base:1 ↔ roja-v1-3DP-lipo-box:1
## Named parameters: d159_d51 = 0 mm, d160_d52 = 0 mm, d161_d53 = 0 mm, d165_d57 = 0 mm, d166_d58 = 0 mm, d167_d59 = 0 mm, d168_d60 = 0 mm, d176_d40 = 0 mm, d177_d41 = 0 mm, d178_d5 = 5 mm
